# Autodesk Inventor assembly: WCP-0199
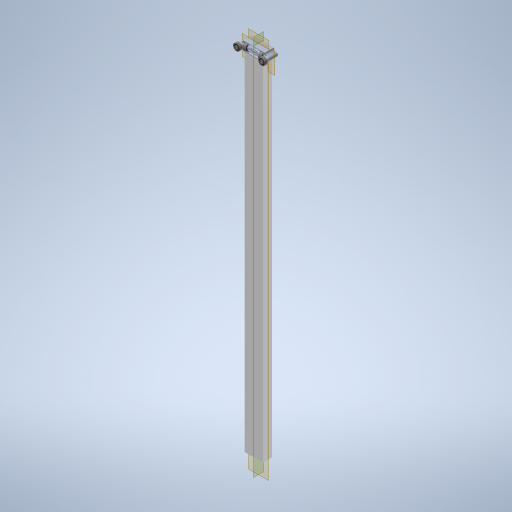
[picture p0: Inventor's stored thumbnail of the model, 512x512]
Saved by Autodesk Inventor 2023.4 (Build 274418000, 418)
## iProperties
Created: 2022-01-07
Part Number: WCP-0199
Description: STEP AP214
Document SubType Name: Assembly
Designer: mavericks
Sending System: SolidWorks 2020
Preprocessor: SwSTEP 2.0
Title: WCP-0199.step
Revision Number: ANY
## Documents named in this file (9)
- C:\Users\mavericks\Documents\Robotics\GitHub\2025-ReefScape---CAD\COMMON PARTS\WCP Elevator parts\WCP-0199\WCP-0199.iam
- C:\Users\mavericks\Documents\Robotics\GitHub\2025-ReefScape---CAD\COMMON PARTS\WCP Elevator parts\WCP-0199\WCP-0199-001 Rev2.ipt
- C:\Users\mavericks\Documents\Robotics\GitHub\2025-ReefScape---CAD\COMMON PARTS\WCP Elevator parts\WCP-0199\WCP-0199-004 Rev2.ipt
- C:\Users\mavericks\Documents\Robotics\GitHub\2025-ReefScape---CAD\COMMON PARTS\WCP Elevator parts\WCP-0199\WCP-0199-003 Rev2_0.750 Bearing.ipt
- C:\Users\mavericks\Documents\Robotics\GitHub\2025-ReefScape---CAD\COMMON PARTS\WCP Elevator parts\WCP-0199\WCP-0199-007 Rev2_0.750 Bearing.ipt
- C:\Users\mavericks\Documents\Robotics\GitHub\2025-ReefScape---CAD\COMMON PARTS\WCP Elevator parts\WCP-0199\WCP-0474 Rev1.ipt
- C:\Users\mavericks\Documents\Robotics\GitHub\2025-ReefScape---CAD\COMMON PARTS\WCP Elevator parts\WCP-0199\WCP-0212_0_250_radial_bearing.ipt
- C:\Users\mavericks\Documents\Robotics\GitHub\2025-ReefScape---CAD\COMMON PARTS\WCP Elevator parts\WCP-0199\WCP-0039 Rev1.ipt
- C:\Users\mavericks\Documents\Robotics\GitHub\2025-ReefScape---CAD\Elevator\EL2\EL2-001.ipt
## Components (17 placed, 17 different names)
1. WCP-0199-001 Rev2_1 — Flush:2, Mate:2, Mate:3
2. WCP-0199-004 Rev2_2
3. WCP-0199-003 Rev2_0.750 Bearing_3
4. WCP-0199-007 Rev2_0.750 Bearing_4
5. WCP-0199-007 Rev2_0.750 Bearing_5
6. WCP-0199-003 Rev2_0.750 Bearing_6
7. WCP-0474 Rev1_7
8. WCP-0474 Rev1_8
9. WCP-0212_0_250_radial_bearing_9
10. WCP-0212_0_250_radial_bearing_10
11. WCP-0212_0_250_radial_bearing_11
12. WCP-0212_0_250_radial_bearing_12
13. WCP-0039 Rev1_13
14. WCP-0039 Rev1_14
15. WCP-0039 Rev1_15
16. WCP-0039 Rev1_16
17. EL2-001:1 — Flush:2, Mate:2, Mate:3
## Relationships (3: Mate 2, Flush 1)
- Flush:2: WCP-0199-001 Rev2_1 ↔ EL2-001:1
- Mate:2: WCP-0199-001 Rev2_1 ↔ EL2-001:1
- Mate:3: WCP-0199-001 Rev2_1 ↔ EL2-001:1
